# Autodesk Inventor assembly: LEFT REAR BUKHEAD
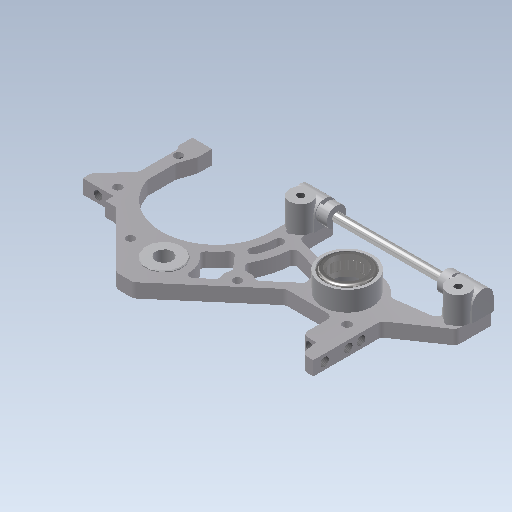
[picture p0: Inventor's stored thumbnail of the model, 512x512]
Saved by Autodesk Inventor 2020 (Build 240168000, 168)
## iProperties
Created: 2015-04-18
Part Number: LEFT REAR BUKHEAD
Document SubType Name: Assembly
Designer: Station9
Author: Station9
## Documents named in this file (10)
- C:\Users\0x6f736f646f\Downloads\rc-car-16.snapshot.3\LEFT REAR BUKHEAD.iam
- C:\Users\0x6f736f646f\Downloads\rc-car-16.snapshot.3\500-171.ipt
- C:\Users\0x6f736f646f\Downloads\rc-car-16.snapshot.3\500-172.ipt
- C:\Users\0x6f736f646f\Downloads\rc-car-16.snapshot.3\500-168.ipt
- C:\Users\0x6f736f646f\Downloads\rc-car-16.snapshot.3\500-160.ipt
- C:\Users\0x6f736f646f\Downloads\rc-car-16.snapshot.3\500-169.ipt
- C:\Users\0x6f736f646f\Downloads\rc-car-16.snapshot.3\500-136.ipt
- C:\Users\0x6f736f646f\Downloads\rc-car-16.snapshot.3\500-141.ipt
- C:\Users\0x6f736f646f\Downloads\rc-car-16.snapshot.3\ISO 3245 - 21 D - 12 x 16 x 7(1) I.ipt
- C:\Users\0x6f736f646f\Downloads\rc-car-16.snapshot.3\500-138.ipt
## Components (11 placed, 9 different names)
1. 500-171:1 — Mate:2, Mate:4, Mate:6, Mate:9
2. 500-172:1 — Mate:1, Mate:3, Mate:5, Mate:7, Mate:15
3. 500-168:1 — Mate:8, Mate:9, Mate:11, Angle:1
4. 500-160:1 — Mate:10, Mate:11, Angle:1
5. 500-138:1
6. 500-169:1 — Mate:5, Mate:6, Mate:7, Mate:8, Mate:10, Mate:13, Mate:14
7. 500-136:1 — Insert:3, Insert:4
8. 500-141:1 — Mate:1, Mate:2, Mate:3, Mate:4, Insert:3
9. 500-168:2 — Mate:13, Mate:15
10. 500-160:2 — Mate:14
11. ISO 3245 (I) 21 D - 12 x 16 x 7:1 — Insert:4
## Relationships (20: Mate 15, Insert 3, Angle 2)
- Mate:1: 500-172:1 ↔ 500-141:1
- Mate:2: 500-171:1 ↔ 500-141:1
- Mate:3: 500-172:1 ↔ 500-141:1
- Mate:4: 500-171:1 ↔ 500-141:1
- Mate:5: 500-172:1 ↔ 500-169:1
- Mate:6: 500-171:1 ↔ 500-169:1
- Mate:7: 500-172:1 ↔ 500-169:1
- [Insert]: 500-138:1 ↔ 500-141:1
- Mate:8: 500-168:1 ↔ 500-169:1
- Mate:9: 500-171:1 ↔ 500-168:1
- Mate:10: 500-160:1 ↔ 500-169:1
- Mate:11: 500-168:1 ↔ 500-160:1
- Angle:1 (0 deg): 500-168:1 ↔ 500-160:1
- [Mate]: 500-168:2 ↔ 500-160:2
- [Angle] (0 deg): 500-168:2 ↔ 500-160:2
- Mate:13: 500-169:1 ↔ 500-168:2
- Mate:14: 500-169:1 ↔ 500-160:2
- Mate:15: 500-172:1 ↔ 500-168:2
- Insert:3: 500-136:1 ↔ 500-141:1
- Insert:4: 500-136:1 ↔ ISO 3245 (I) 21 D - 12 x 16 x 7:1
## Named parameters: d20_d18 = 0 mm, d21_d19 = 0 deg
